# Autodesk Inventor assembly: JH_Greifer_Scheibe
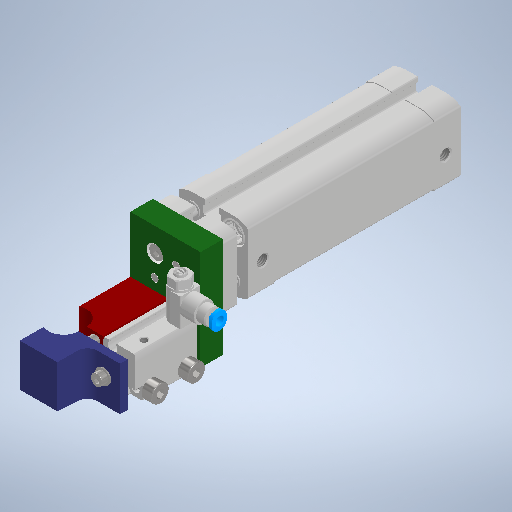
[picture p0: Inventor's stored thumbnail of the model, 512x512]
Saved by Autodesk Inventor 2025.1 (Build 291241000, 241)
## iProperties
Created: 2025-06-16
Part Number: JH_Greifer_Scheibe
Document SubType Name: Assembly
Designer: Jakob
Author: Jakob
## Documents named in this file (16)
- C:\Users\Erik\Erik\Hochschule\3. Semester\CAD\CAD-Paspa\Useless Box\Eigene Bauteile\JH_Greifer_Unterlegscheibe\Eigene Bauteile\JH_Greifer_Scheibe.iam
- C:\Users\Erik\Erik\Hochschule\3. Semester\CAD\CAD-Paspa\Useless Box\Eigene Bauteile\JH_Greifer_Unterlegscheibe\Eigene Bauteile\JH_int_Greiferkoerper.ipt
- C:\Users\Erik\Erik\Hochschule\3. Semester\CAD\CAD-Paspa\Useless Box\Eigene Bauteile\JH_Greifer_Unterlegscheibe\Eigene Bauteile\JH_int_Greiferkoerper_Gegenstueck.ipt
- C:\Users\Erik\Erik\Hochschule\3. Semester\CAD\CAD-Paspa\Useless Box\Eigene Bauteile\JH_Greifer_Unterlegscheibe\Kaufteile\AIS2024\5267300 AEN-S-6-5-I-A---(0_high).iam
- C:\Users\Erik\Erik\Hochschule\3. Semester\CAD\CAD-Paspa\Useless Box\Standart Bauteile\DIN 125 - A 2,7.ipt
- C:\Users\Erik\Erik\Hochschule\3. Semester\CAD\CAD-Paspa\Useless Box\Standart Bauteile\DIN EN ISO 4762 - M2,5 x 5.ipt
- C:\Users\Erik\Erik\Hochschule\3. Semester\CAD\CAD-Paspa\Useless Box\Standart Bauteile\DIN EN ISO 2338 - 4 h8 x 14.ipt
- C:\Users\Erik\Erik\Hochschule\3. Semester\CAD\CAD-Paspa\Useless Box\Eigene Bauteile\JH_Greifer_Unterlegscheibe\Kaufteile\AIS2024\Unterlegscheibe.ipt
- C:\Users\Erik\Erik\Hochschule\3. Semester\CAD\CAD-Paspa\Useless Box\Eigene Bauteile\JH_Greifer_Unterlegscheibe\Kaufteile\Drosselrückschlagventil\175043 GRLZ-M3-QS-3.ipt
- C:\Users\Erik\Erik\Hochschule\3. Semester\CAD\CAD-Paspa\Useless Box\Standart Bauteile\DIN EN ISO 4762 - M4 x 16.ipt
- C:\Users\Erik\Erik\Hochschule\3. Semester\CAD\CAD-Paspa\Useless Box\Eigene Bauteile\JH_Greifer_Unterlegscheibe\Kaufteile\Führungszylinder\AIS2024\537123 ADNGF-12-50-P-A---(0).iam
- C:\Users\Erik\Erik\Hochschule\3. Semester\CAD\CAD-Paspa\Useless Box\Eigene Bauteile\JH_Greifer_Unterlegscheibe\Eigene Bauteile\JH_int_Adapterplatte.ipt
- C:\Users\Erik\Erik\Hochschule\3. Semester\CAD\CAD-Paspa\Useless Box\Standart Bauteile\DIN EN ISO 4762 - M3 x 5.ipt
- C:\Users\Erik\Erik\Hochschule\3. Semester\CAD\CAD-Paspa\Useless Box\Standart Bauteile\DIN EN ISO 2338 - 3 h8 x 10.ipt
- C:\Users\Erik\Erik\Hochschule\3. Semester\CAD\CAD-Paspa\Useless Box\Standart Bauteile\DIN EN ISO 2338 - 3 h8 x 14.ipt
- C:\Users\Erik\Erik\Hochschule\3. Semester\CAD\CAD-Paspa\Useless Box\Standart Bauteile\DIN EN ISO 4762 - M3 x 10.ipt
## Components (20 placed, 15 different names)
1. JH_int_Greiferkoerper:1 — Flush:1, Flush:2, Flush:3, Mate:2, Mate:3, Mate:4, Mate:9, Mate:10, Mate:11, Mate:12, Mate:28, Mate:29, Mate:30
2. JH_int_Greiferkoerper_Gegenstueck:1 — Mate:1, Flush:4, Flush:5, Mate:5, Flush:6, Mate:20
3. 5267300 AEN-S-6-5-I-A---(0_high):1 [sub-assembly] — Mate:2, Mate:3, Mate:4, Flush:5, Mate:6, Mate:7, Mate:18, Mate:19, Mate:24, Mate:25, Mate:26, Mate:27
4. DIN 125 - A 2,7:1 — Mate:5, Mate:6, Mate:8
5. DIN EN ISO 4762 - M2,5 x 5:1 — Mate:7, Mate:8
6. DIN EN ISO 2338 - 4 h8 x 14:1 — Mate:9, Mate:10
7. DIN EN ISO 2338 - 4 h8 x 14:2 — Mate:11, Mate:12
8. DIN 9021 2,7:1 — Mate:20
9. 175043 GRLZ-M3-QS-3:1 — Angle:1, Mate:18, Mate:19
10. DIN EN ISO 4762 - M4 x 16:1 — Mate:24, Mate:27
11. DIN EN ISO 4762 - M4 x 16:2 — Mate:25, Mate:26
12. 537123 ADNGF-12-50-P-A---(0):1 [sub-assembly] — Mate:31, Mate:32, Mate:33
13. JH_int_Adapterplatte:1 — Mate:28, Mate:29, Mate:30, Mate:31, Mate:32, Mate:33, Mate:34, Mate:35, Mate:36, Mate:37, Mate:38, Flush:7, Mate:39, Mate:40, Flush:8, Flush:9, Mate:41, Mate:42, Mate:43, Mate:44
14. DIN EN ISO 4762 - M3 x 5:1 — Mate:34, Mate:36
15. DIN EN ISO 4762 - M3 x 5:2 — Mate:35, Mate:37
16. DIN EN ISO 2338 - 3 h8 x 10:1 — Mate:38, Flush:7
17. DIN EN ISO 2338 - 3 h8 x 14:1 — Mate:40, Flush:8
18. DIN EN ISO 2338 - 3 h8 x 14:2 — Mate:39, Flush:9
19. DIN EN ISO 4762 - M3 x 10:1 — Mate:42, Mate:44
20. DIN EN ISO 4762 - M3 x 10:2 — Mate:41, Mate:43
## Relationships (46: Mate 36, Flush 9, Angle 1)
- Flush:1: JH_int_Greiferkoerper:1
- Flush:2: JH_int_Greiferkoerper:1
- Flush:3: JH_int_Greiferkoerper:1
- Mate:1: JH_int_Greiferkoerper_Gegenstueck:1
- Flush:4: JH_int_Greiferkoerper_Gegenstueck:1
- Mate:2: JH_int_Greiferkoerper:1 ↔ 5267300 AEN-S-6-5-I-A---(0_high):1
- Mate:3: JH_int_Greiferkoerper:1 ↔ 5267300 AEN-S-6-5-I-A---(0_high):1
- Mate:4: JH_int_Greiferkoerper:1 ↔ 5267300 AEN-S-6-5-I-A---(0_high):1
- Flush:5: JH_int_Greiferkoerper_Gegenstueck:1 ↔ 5267300 AEN-S-6-5-I-A---(0_high):1
- Mate:5: JH_int_Greiferkoerper_Gegenstueck:1 ↔ DIN 125 - A 2,7:1
- Mate:6: 5267300 AEN-S-6-5-I-A---(0_high):1 ↔ DIN 125 - A 2,7:1
- Mate:7: 5267300 AEN-S-6-5-I-A---(0_high):1 ↔ DIN EN ISO 4762 - M2,5 x 5:1
- Mate:8: DIN 125 - A 2,7:1 ↔ DIN EN ISO 4762 - M2,5 x 5:1
- Mate:9: JH_int_Greiferkoerper:1 ↔ DIN EN ISO 2338 - 4 h8 x 14:1
- Mate:10: JH_int_Greiferkoerper:1 ↔ DIN EN ISO 2338 - 4 h8 x 14:1
- Mate:11: JH_int_Greiferkoerper:1 ↔ DIN EN ISO 2338 - 4 h8 x 14:2
- Mate:12: JH_int_Greiferkoerper:1 ↔ DIN EN ISO 2338 - 4 h8 x 14:2
- Angle:1 (0 deg): 175043 GRLZ-M3-QS-3:1
- Mate:18: 5267300 AEN-S-6-5-I-A---(0_high):1 ↔ 175043 GRLZ-M3-QS-3:1
- Mate:19: 5267300 AEN-S-6-5-I-A---(0_high):1 ↔ 175043 GRLZ-M3-QS-3:1
- Flush:6 (-2.541 mm): JH_int_Greiferkoerper_Gegenstueck:1
- Mate:20 (7.95 mm): JH_int_Greiferkoerper_Gegenstueck:1 ↔ DIN 9021 2,7:1
- Mate:24: 5267300 AEN-S-6-5-I-A---(0_high):1 ↔ DIN EN ISO 4762 - M4 x 16:1
- Mate:25: 5267300 AEN-S-6-5-I-A---(0_high):1 ↔ DIN EN ISO 4762 - M4 x 16:2
- Mate:26: 5267300 AEN-S-6-5-I-A---(0_high):1 ↔ DIN EN ISO 4762 - M4 x 16:2
- Mate:27: 5267300 AEN-S-6-5-I-A---(0_high):1 ↔ DIN EN ISO 4762 - M4 x 16:1
- Mate:28: JH_int_Greiferkoerper:1 ↔ JH_int_Adapterplatte:1
- Mate:29: JH_int_Greiferkoerper:1 ↔ JH_int_Adapterplatte:1
- Mate:30: JH_int_Greiferkoerper:1 ↔ JH_int_Adapterplatte:1
- Mate:31: 537123 ADNGF-12-50-P-A---(0):1 ↔ JH_int_Adapterplatte:1
- Mate:32: 537123 ADNGF-12-50-P-A---(0):1 ↔ JH_int_Adapterplatte:1
- Mate:33: 537123 ADNGF-12-50-P-A---(0):1 ↔ JH_int_Adapterplatte:1
- Mate:34: JH_int_Adapterplatte:1 ↔ DIN EN ISO 4762 - M3 x 5:1
- Mate:35: JH_int_Adapterplatte:1 ↔ DIN EN ISO 4762 - M3 x 5:2
- Mate:36: JH_int_Adapterplatte:1 ↔ DIN EN ISO 4762 - M3 x 5:1
- Mate:37: JH_int_Adapterplatte:1 ↔ DIN EN ISO 4762 - M3 x 5:2
- Mate:38: JH_int_Adapterplatte:1 ↔ DIN EN ISO 2338 - 3 h8 x 10:1
- Flush:7: JH_int_Adapterplatte:1 ↔ DIN EN ISO 2338 - 3 h8 x 10:1
- Mate:39: JH_int_Adapterplatte:1 ↔ DIN EN ISO 2338 - 3 h8 x 14:2
- Mate:40: JH_int_Adapterplatte:1 ↔ DIN EN ISO 2338 - 3 h8 x 14:1
- Flush:8: JH_int_Adapterplatte:1 ↔ DIN EN ISO 2338 - 3 h8 x 14:1
- Flush:9: JH_int_Adapterplatte:1 ↔ DIN EN ISO 2338 - 3 h8 x 14:2
- Mate:41: JH_int_Adapterplatte:1 ↔ DIN EN ISO 4762 - M3 x 10:2
- Mate:42: JH_int_Adapterplatte:1 ↔ DIN EN ISO 4762 - M3 x 10:1
- Mate:43: JH_int_Adapterplatte:1 ↔ DIN EN ISO 4762 - M3 x 10:2
- Mate:44: JH_int_Adapterplatte:1 ↔ DIN EN ISO 4762 - M3 x 10:1
